# Autodesk Inventor assembly: Gearbox
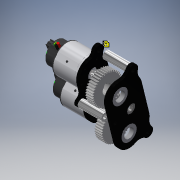
[picture p0: Inventor's stored thumbnail of the model, 180x180]
Saved by Autodesk Inventor 2019.4 (Build 234330000, 330)
## iProperties
Created: 2019-12-11
Part Number: Gearbox
Document SubType Name: Assembly
Designer: admin
Author: admin
## Documents named in this file (12)
- C:\Users\admin\Desktop\FRC 2020 Engineering\GitHub\7738-CAD-prep\Offline CAD\MK3 Gearbox\Gearbox.iam
- C:\Users\admin\Desktop\FRC 2020 Engineering\GitHub\7738-CAD-prep\Swerve Module\Falcon_500_Powered_by_Talon_FX_217-6515.iam
- C:\Users\admin\Desktop\FRC 2020 Engineering\GitHub\7738-CAD-prep\WCD\10T_Steel_Spur_Gear_20_DP_12T_Center_Distance_Falcon_Motor_217-6917.ipt
- C:\Users\admin\Desktop\FRC 2020 Engineering\GitHub\7738-CAD-prep\Offline CAD\MK3 Gearbox\40t_Aluminum_Spur_Gear_20_DP_1_2_Hex_Bore_217-2708.ipt
- C:\Users\admin\Desktop\FRC 2020 Engineering\GitHub\7738-CAD-prep\Offline CAD\MK3 Gearbox\Gearbox\Design Accelerator\Spur Gears1.iam
- C:\Users\admin\Desktop\FRC 2020 Engineering\GitHub\7738-CAD-prep\Butterfly drive\F6800Z 10mm ID Flange.ipt
- C:\Users\admin\Desktop\FRC 2020 Engineering\GitHub\7738-CAD-prep\Offline CAD\MK3 Gearbox\Gearbox Plate 1.ipt
- C:\Users\admin\Desktop\FRC 2020 Engineering\GitHub\7738-CAD-prep\Offline CAD\MK3 Gearbox\Gearbox Plate 2.ipt
- C:\Users\admin\Desktop\FRC 2020 Engineering\GitHub\7738-CAD-prep\Offline CAD\MK3 Gearbox\Shaft Jr.ipt
- C:\Users\admin\Desktop\FRC 2020 Engineering\GitHub\7738-CAD-prep\Offline CAD\F6804.ipt
- C:\Users\admin\Desktop\FRC 2020 Engineering\GitHub\7738-CAD-prep\Offline CAD\MK3 Gearbox\Gearbox\Design Accelerator\Spur Gears2.iam
- C:\Users\admin\Desktop\FRC 2020 Engineering\GitHub\7738-CAD-prep\Offline CAD\Gearbox Spacer.ipt
## Components (17 placed, 10 different names)
1. Falcon_500_Powered_by_Talon_FX_217-6515:1 [sub-assembly] — Mate:5, Mate:6, Mate:16
2. 10T_Steel_Spur_Gear_20_DP_12T_Center_Distance_Falcon_Motor_217-6917:2 — Mate:16, Mate:17
3. 10T_Steel_Spur_Gear_20_DP_12T_Center_Distance_Falcon_Motor_217-6917:3 — Mate:15, Mate:18
4. 40t_Aluminum_Spur_Gear_20_DP_1_2_Hex_Bore_217-2708:1 — Mate:21, Mate:22, Mate:38, Mate:39
5. Spur Gears:1 [sub-assembly] — Mate:29, Flush:2, Mate:38, Mate:39
6. Gearbox Plate 1:1 — Flush:1, Mate:5, Mate:6, Mate:7, Mate:8, Mate:17, Mate:18, Mate:19, Mate:20, Mate:26, Mate:36, Mate:37
7. Gearbox Plate 2:1 — Flush:1, Mate:9, Mate:10, Mate:11, Mate:12, Mate:13, Mate:14, Mate:26, Mate:32, Mate:33, Mate:34, Mate:35
8. F6800Z 10mm ID Flange:2 — Mate:9, Mate:10, Mate:25
9. Shaft Jr:1 — Mate:23, Mate:24, Mate:25
10. Falcon_500_Powered_by_Talon_FX_217-6515:2 [sub-assembly] — Mate:7, Mate:8, Mate:15
11. F6804:1 — Mate:11, Mate:12, Mate:30
12. F6804:2 — Mate:13, Mate:14, Mate:29
13. F6800Z 10mm ID Flange:3 — Mate:19, Mate:20, Mate:21, Mate:22, Mate:23, Mate:24
14. Spur Gears:2 [sub-assembly] — Mate:30, Flush:2
15. Gearbox Spacer:1 — Mate:32, Mate:33
16. Gearbox Spacer:2 — Mate:34, Mate:35
17. Gearbox Spacer:3 — Mate:36, Mate:37
## Relationships (34: Mate 32, Flush 2)
- Flush:1: Gearbox Plate 1:1 ↔ Gearbox Plate 2:1
- Mate:5: Falcon_500_Powered_by_Talon_FX_217-6515:1 ↔ Gearbox Plate 1:1
- Mate:6: Falcon_500_Powered_by_Talon_FX_217-6515:1 ↔ Gearbox Plate 1:1
- Mate:7: Gearbox Plate 1:1 ↔ Falcon_500_Powered_by_Talon_FX_217-6515:2
- Mate:8: Gearbox Plate 1:1 ↔ Falcon_500_Powered_by_Talon_FX_217-6515:2
- Mate:9: Gearbox Plate 2:1 ↔ F6800Z 10mm ID Flange:2
- Mate:10 (0.1 mm): Gearbox Plate 2:1 ↔ F6800Z 10mm ID Flange:2
- Mate:11 (0.1 mm): Gearbox Plate 2:1 ↔ F6804:1
- Mate:12: Gearbox Plate 2:1 ↔ F6804:1
- Mate:13 (0.1 mm): Gearbox Plate 2:1 ↔ F6804:2
- Mate:14: Gearbox Plate 2:1 ↔ F6804:2
- Mate:15: 10T_Steel_Spur_Gear_20_DP_12T_Center_Distance_Falcon_Motor_217-6917:3 ↔ Falcon_500_Powered_by_Talon_FX_217-6515:2
- Mate:16: Falcon_500_Powered_by_Talon_FX_217-6515:1 ↔ 10T_Steel_Spur_Gear_20_DP_12T_Center_Distance_Falcon_Motor_217-6917:2
- Mate:17 (1 mm): 10T_Steel_Spur_Gear_20_DP_12T_Center_Distance_Falcon_Motor_217-6917:2 ↔ Gearbox Plate 1:1
- Mate:18 (1 mm): 10T_Steel_Spur_Gear_20_DP_12T_Center_Distance_Falcon_Motor_217-6917:3 ↔ Gearbox Plate 1:1
- Mate:19 (0.1 mm): Gearbox Plate 1:1 ↔ F6800Z 10mm ID Flange:3
- Mate:20: Gearbox Plate 1:1 ↔ F6800Z 10mm ID Flange:3
- Mate:21 (5 mm): 40t_Aluminum_Spur_Gear_20_DP_1_2_Hex_Bore_217-2708:1 ↔ F6800Z 10mm ID Flange:3
- Mate:22: 40t_Aluminum_Spur_Gear_20_DP_1_2_Hex_Bore_217-2708:1 ↔ F6800Z 10mm ID Flange:3
- Mate:23 (0.1 mm): Shaft Jr:1 ↔ F6800Z 10mm ID Flange:3
- Mate:24: Shaft Jr:1 ↔ F6800Z 10mm ID Flange:3
- Mate:25: F6800Z 10mm ID Flange:2 ↔ Shaft Jr:1
- Mate:26 (65 mm): Gearbox Plate 1:1 ↔ Gearbox Plate 2:1
- Mate:29: Spur Gears:1 ↔ F6804:2
- Mate:30: F6804:1 ↔ Spur Gears:2
- Flush:2: Spur Gears:1 ↔ Spur Gears:2
- Mate:32: Gearbox Plate 2:1 ↔ Gearbox Spacer:1
- Mate:33 (0.2 mm): Gearbox Plate 2:1 ↔ Gearbox Spacer:1
- Mate:34: Gearbox Plate 2:1 ↔ Gearbox Spacer:2
- Mate:35 (0.2 mm): Gearbox Plate 2:1 ↔ Gearbox Spacer:2
- Mate:36: Gearbox Plate 1:1 ↔ Gearbox Spacer:3
- Mate:37 (0.2 mm): Gearbox Plate 1:1 ↔ Gearbox Spacer:3
- Mate:38: 40t_Aluminum_Spur_Gear_20_DP_1_2_Hex_Bore_217-2708:1 ↔ Spur Gears:1
- Mate:39 (11 mm): 40t_Aluminum_Spur_Gear_20_DP_1_2_Hex_Bore_217-2708:1 ↔ Spur Gears:1
